# Autodesk Inventor assembly: Assembly_Guinardia_V1
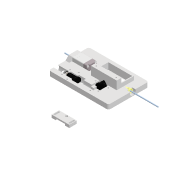
[picture p0: Inventor's stored thumbnail of the model, 180x180]
Saved by Autodesk Inventor 2022 (Build 260153000, 153)
## iProperties
Created: 2022-04-18
Part Number: Assembly_Guinardia_V1
Document SubType Name: Assembly
Designer: Prakash Lab
Author: Prakash Lab
## Documents named in this file (10)
- C:\Users\UC2\Documents\GitHub\Guinardia\INVENTOR\Assembly_Guinardia_V1.iam
- C:\Users\UC2\Documents\GitHub\Guinardia\INVENTOR\00_NEMA8.ipt
- C:\Users\UC2\Documents\GitHub\Guinardia\INVENTOR\00_CCTV_lens_M12_25mm_5mp.ipt
- C:\Users\UC2\Documents\GitHub\Guinardia\INVENTOR\00_coverslip_24x50mm.ipt
- C:\Users\UC2\Documents\GitHub\Guinardia\INVENTOR\00_PipetteTip200ul-1.ipt
- C:\Users\UC2\Documents\GitHub\Guinardia\INVENTOR\00_FEP_tube_2.2x0.5mm.ipt
- C:\Users\UC2\Documents\GitHub\Guinardia\INVENTOR\10_LED_cylnderlensmount.ipt
- C:\Users\UC2\Documents\GitHub\Guinardia\INVENTOR\10_Wellplate_base_v1.ipt
- C:\Users\UC2\Documents\GitHub\Guinardia\INVENTOR\00_SM05FC2-Step.ipt
- C:\Users\UC2\Documents\GitHub\Guinardia\INVENTOR\00_HuaweiP30_Telelens_prismonly.ipt
## Components (12 placed, 9 different names)
1. 10_Wellplate_base_v1:1 — Mate:1, Mate:2, Mate:3, Mate:4, Mate:5, Flush:1, Mate:10, Flush:2, Mate:11, Mate:12, Einfügen:2, Winkel:1, Winkel:2, Passend:15, Fluchtend:3
2. 00_CCTV_lens_M12_25mm_5mp:1 — Mate:6, Flush:1, Passend:14, Passend:17, Passend:18
3. 00_coverslip_24x50mm:1 — Mate:1, Mate:2, Mate:3, Mate:7, Mate:13
4. 00_PipetteTip200ul-1:2 — Mate:9, Flush:2
5. 00_FEP_tube_2.2x0.5mm:1 — Mate:4, Mate:5, Mate:8, Mate:9, Mate:7
6. 00_PipetteTip200ul-1:3 — Mate:8, Mate:6, Mate:10
7. 00_coverslip_24x50mm:2 — Mate:11, Mate:12, Mate:13
8. 00_NEMA8:1 — Einfügen:2, Winkel:1
9. 00_HuaweiP30_Telelens_prismonly:1 — Passend:16, Passend:17, Passend:18
10. 10_LED_cylnderlensmount:1
11. 00_SM05FC2-Step:1 — Passend:14, Winkel:2, Passend:15, Fluchtend:3, Passend:16, Einfügen:3
12. 00_CCTV_lens_M12_25mm_5mp:2 — Einfügen:3
## Relationships (25: Mate 18, Flush 3, Insert 2, Angle 2)
- Mate:1: 10_Wellplate_base_v1:1 ↔ 00_coverslip_24x50mm:1
- Mate:2: 10_Wellplate_base_v1:1 ↔ 00_coverslip_24x50mm:1
- Mate:3: 10_Wellplate_base_v1:1 ↔ 00_coverslip_24x50mm:1
- Mate:4 (-6 mm): 10_Wellplate_base_v1:1 ↔ 00_FEP_tube_2.2x0.5mm:1
- Mate:5: 10_Wellplate_base_v1:1 ↔ 00_FEP_tube_2.2x0.5mm:1
- Mate:8: 00_FEP_tube_2.2x0.5mm:1 ↔ 00_PipetteTip200ul-1:3
- Mate:9: 00_PipetteTip200ul-1:2 ↔ 00_FEP_tube_2.2x0.5mm:1
- Mate:6: 00_CCTV_lens_M12_25mm_5mp:1 ↔ 00_PipetteTip200ul-1:3
- Flush:1: 10_Wellplate_base_v1:1 ↔ 00_CCTV_lens_M12_25mm_5mp:1
- Mate:7 (3 mm): 00_coverslip_24x50mm:1 ↔ 00_FEP_tube_2.2x0.5mm:1
- Mate:10 (4 mm): 10_Wellplate_base_v1:1 ↔ 00_PipetteTip200ul-1:3
- Flush:2 (5 mm): 10_Wellplate_base_v1:1 ↔ 00_PipetteTip200ul-1:2
- Mate:11: 10_Wellplate_base_v1:1 ↔ 00_coverslip_24x50mm:2
- Mate:12: 10_Wellplate_base_v1:1 ↔ 00_coverslip_24x50mm:2
- Mate:13: 00_coverslip_24x50mm:1 ↔ 00_coverslip_24x50mm:2
- Einfügen:2 [Insert]: 10_Wellplate_base_v1:1 ↔ 00_NEMA8:1
- Winkel:1 [Angle] (0 deg): 10_Wellplate_base_v1:1 ↔ 00_NEMA8:1
- Passend:14 [Mate]: 00_CCTV_lens_M12_25mm_5mp:1 ↔ 00_SM05FC2-Step:1
- Winkel:2 [Angle] (180 deg): 10_Wellplate_base_v1:1 ↔ 00_SM05FC2-Step:1
- Passend:15 [Mate] (-15 mm): 10_Wellplate_base_v1:1 ↔ 00_SM05FC2-Step:1
- Fluchtend:3 [Flush] (20 mm): 10_Wellplate_base_v1:1 ↔ 00_SM05FC2-Step:1
- Passend:16 [Mate]: 00_HuaweiP30_Telelens_prismonly:1 ↔ 00_SM05FC2-Step:1
- Passend:17 [Mate]: 00_CCTV_lens_M12_25mm_5mp:1 ↔ 00_HuaweiP30_Telelens_prismonly:1
- Passend:18 [Mate]: 00_CCTV_lens_M12_25mm_5mp:1 ↔ 00_HuaweiP30_Telelens_prismonly:1
- Einfügen:3 [Insert] (5 mm): 00_SM05FC2-Step:1 ↔ 00_CCTV_lens_M12_25mm_5mp:2
